# Autodesk Inventor assembly: main
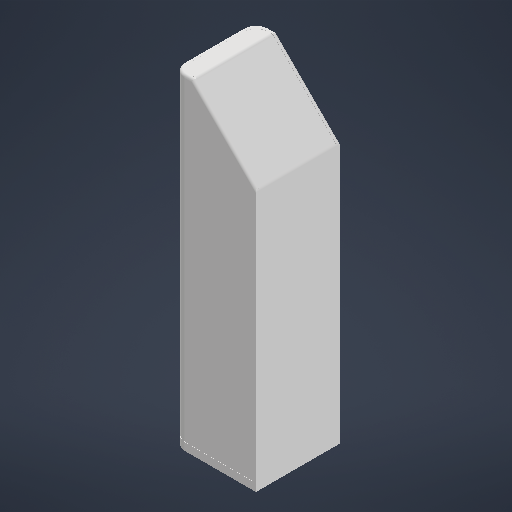
[picture p0: Inventor's stored thumbnail of the model, 512x512]
Saved by Autodesk Inventor 2027 (Build 310192060, 192F)
## iProperties
Created: 2026-07-05
Part Number: main
Document SubType Name: Assembly
Designer: User
Author: User
## Documents named in this file (3)
- G:\Github\Alkomaster\Alkomaster\Hardware\main.iam
- G:\Github\Alkomaster\Alkomaster\Hardware\Parts\Frame.ipt
- G:\Github\Alkomaster\Alkomaster\Hardware\Parts\bottom_frame.ipt
## Components (2 placed, 2 different names)
1. Frame:1 — przesuwne:1
2. bottom_frame:1 — przesuwne:1
## Relationships (1: TranslationJoint 1)
- przesuwne:1 [TranslationJoint]: Frame:1 ↔ bottom_frame:1
